# Autodesk Inventor assembly: HHS25
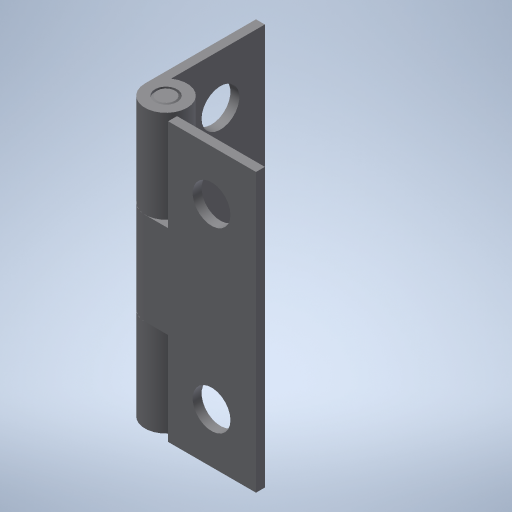
[picture p0: Inventor's stored thumbnail of the model, 512x512]
Saved by Autodesk Inventor 2024.2 (Build 282272000, 272)
## iProperties
Category: PARTsolutions
Company: MISUMI
Created: 2024-01-05
Part Number: HHS25
Description: HHS-Butt Hinges
Vendor: MISUMI
Document SubType Name: Assembly
Designer: psAdmin
Manufacturer: MISUMI
Mass: 0.590722 g
Surface Area: 15.2968 cm^2
Volume: 0.590722 cm^3
Density: 1 g/cm^3
Catalog Web Link: https://jp.misumi-ec.com/vona2/detail/110300524240/?ProductCode=HHS25
PSOL_IDENT_0: {$CADENAS_DATA/23d-libs/misumi/metric/43_levers_knobs/assemblies_hhs/hhs_asmtab.prj},156 {VTYP=3D},{
PSOL_IDENT_1: STYP=ASSTAB},{NB=HHS25},{LINA=HHS25},{NN=HHS},{DATE=04.06.2021 08:38:48},{GEOMDATE=19.02.2008},{VERS
PSOL_IDENT_2: ION=},{LINEID=10},{WBVAR=LS},{WBNUMERIC=LS}  {NB=HHS25},{LINA=HHS25},{KT=DUMMY},{PN=HHS25},{MAT=SUS3
PSOL_IDENT_3: 04(304 Stainless Steel)(1.4301_X5CrNi18-10)},{NO=25},{LS=25},{L111=25,30,40,50,65,75,90,100},{SHPNO=
PSOL_IDENT_4: A},{W=20},{W1=12},{W2=0},{L1=16},{L2=0},{L3=0},{C=2},{C1=3.8},{TT=0.8},{DD=3.4},{NOD=3},{AL=9.8},{WT=
PSOL_IDENT_5: 6},{LL=20.5},{LLY=4.5},{PPATH=hhs_asmtpl.prj}
NB: HHS25
NN: HHS
NT: Butt Hinges
NBSYN: $PN.
LINA: HHS25
CATALOG: Misumi
PN: HHS25
MAT: 304 Stainless Steel
NO: 25
LS: 25
SHPNO: A
W: 20
W1: 12
W2: 0
L1: 16
L2: 0
L3: 0
C: 2
C1: 3.8
TT: 0.8
DD: 3.4
NOD: 3
AL: 9.8
WT: 6
SUPPLIER: MISUMI
ARTICLENO: HHS25
BOMINFO: HHS25
CREATOR: CADENAS GmbH
Title: HHS25
Author: Cadenas PARTsolutions
Comments: Butt Hinges
## Documents named in this file (4)
- C:\Users\masato\OneDrive - Chiba Institute of Technology\CIT Brains\RoboCup2024\Mechanic\SUSTAINA-OP2\NativeFiles\Boby\COTS\MisumiComponents\HHS25.iam
- C:\Users\masato\OneDrive - Chiba Institute of Technology\CIT Brains\RoboCup2024\Mechanic\SUSTAINA-OP2\NativeFiles\Boby\COTS\MisumiComponents\HHS25-LEAF1.ipt
- C:\Users\masato\OneDrive - Chiba Institute of Technology\CIT Brains\RoboCup2024\Mechanic\SUSTAINA-OP2\NativeFiles\Boby\COTS\MisumiComponents\HHS25-LEAF2.ipt
- C:\Users\masato\OneDrive - Chiba Institute of Technology\CIT Brains\RoboCup2024\Mechanic\SUSTAINA-OP2\NativeFiles\Boby\COTS\MisumiComponents\HHS25-PIN.ipt
## Components (3 placed, 3 different names)
1. HHS25-LEAF1:1 — to_leaf2_XY@1 <-> to_leaf1_XY@2, to_leaf2_Z@1 <-> to_leaf1_Z@2, to_leaf2_XY@1 <-> to_leaf_XY@3, to_leaf2_Z@1 <-> to_leaf_Z@3, to_leaf2_YZ@1 <-> to_leaf_YZ@3, Angle:2
2. HHS25-LEAF2:1 — to_leaf2_XY@1 <-> to_leaf1_XY@2, to_leaf2_Z@1 <-> to_leaf1_Z@2, Angle:2
3. HHS25-PIN:1 — to_leaf2_XY@1 <-> to_leaf_XY@3, to_leaf2_Z@1 <-> to_leaf_Z@3, to_leaf2_YZ@1 <-> to_leaf_YZ@3
## Relationships (6: Flush 2, Mate 2, Angle 2)
- to_leaf2_XY@1 <-> to_leaf1_XY@2 [Flush]: HHS25-LEAF1:1 ↔ HHS25-LEAF2:1
- to_leaf2_Z@1 <-> to_leaf1_Z@2 [Mate]: HHS25-LEAF1:1 ↔ HHS25-LEAF2:1
- to_leaf2_XY@1 <-> to_leaf_XY@3 [Flush]: HHS25-LEAF1:1 ↔ HHS25-PIN:1
- to_leaf2_Z@1 <-> to_leaf_Z@3 [Mate]: HHS25-LEAF1:1 ↔ HHS25-PIN:1
- to_leaf2_YZ@1 <-> to_leaf_YZ@3 [Angle] (0 deg): HHS25-LEAF1:1 ↔ HHS25-PIN:1
- Angle:2 (90 deg): HHS25-LEAF1:1 ↔ HHS25-LEAF2:1
